# Autodesk Inventor assembly: Сборка1
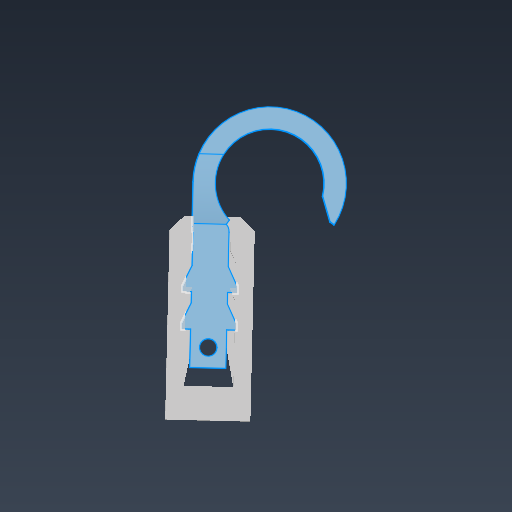
[picture p0: Inventor's stored thumbnail of the model, 512x512]
Saved by Autodesk Inventor 2025 (Build 290162000, 162)
## iProperties
Created: 2025-02-20
Part Number: Сборка1
Document SubType Name: Assembly
Designer: Phantom
Author: Phantom
## Documents named in this file (3)
- C:\Users\GameHD\Desktop\Phantom 16950\Сборка1.iam
- C:\Users\GameHD\Desktop\Phantom 16950\встав для крюка.ipt
- C:\Users\GameHD\Desktop\Phantom 16950\крюк старый.ipt
## Components (2 placed, 2 different names)
1. встав для крюка:1 — Совмещение:1
2. крюк старый:1 — Совмещение:1
## Relationships (1: Mate 1)
- Совмещение:1 [Mate]: встав для крюка:1 ↔ крюк старый:1
